# Autodesk Inventor assembly: Lamp_link
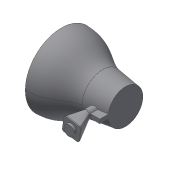
[picture p0: Inventor's stored thumbnail of the model, 180x180]
Saved by Autodesk Inventor 2018 (Build 220112000, 112)
## iProperties
Created: 2019-11-23
Part Number: Lamp_link
Document SubType Name: Assembly
Designer: Clevo
Author: Clevo
## Documents named in this file (3)
- E:\RobotArm\Software\URDF_Files\Lamp_link.iam
- E:\RobotArm\Software\URDF_Files\Lamp_Shade.ipt
- E:\RobotArm\Software\URDF_Files\test_tip.ipt
## Components (2 placed, 2 different names)
1. Lamp_Shade:1 — Mate:1, Mate:2
2. test_tip:1 — Mate:1, Mate:2
## Relationships (2: Mate 2)
- Mate:1: Lamp_Shade:1 ↔ test_tip:1
- Mate:2: Lamp_Shade:1 ↔ test_tip:1
